# Autodesk Inventor assembly: COMPONENTS
(part 3 of 3)
701. RESC1005X35N_R198:1
702. RESC1005X35N_R199:1
703. RESC1005X35N_R200:1
704. RESC1005X35N_R155:1
705. RESC1005X35N_R156:1
706. RESC1005X35N_R225:1
707. RESC1005X35N_R228:1
708. RESC1005X35N_R229:1
709. RESC1005X35N_R230:1
710. RESC1005X35N_R231:1
711. RESC1005X35N_R232:1
712. RESC1005X35N_R233:1
713. RESC1005X35N_R234:1
714. RESC1005X35N_R168:1
715. RESC1005X35N_R181:1
716. RESC1005X35N_R17:1
717. RESC1005X35N_R18:1
718. RESC1005X35N_R37:1
719. RESC1005X35N_R38:1
720. RESC1005X35N_R57:1
721. RESC1005X35N_R58:1
722. RESC1005X35N_R19:1
723. RESC1005X35N_R39:1
724. RESC1005X35N_R59:1
725. RESC1005X35N_R20:1
726. RESC1005X35N_R40:1
727. RESC1005X35N_R60:1
728. RESC1005X35N_R209:1
729. RESC1005X35N_R220:1
730. RESC1005X35N_R61:1
731. RESC1005X35N_R65:1
732. RESC1005X35N_R67:1
733. RESC1005X35N_R62:1
734. RESC1005X35N_R64:1
735. RESC1005X35N_R63:1
736. RESC1005X35N_R66:1
737. RESC1005X35N_R70:1
738. RESC1005X35N_R71:1
739. RESC1005X35N_R72:1
740. RESC1005X35N_R73:1
741. RESC1005X35N_R75:1
742. RESC1005X35N_R76:1
743. RESC1005X35N_R77:1
744. RESC1005X35N_R91:1
745. RESC1005X35N_R92:1
746. RESC1005X35N_R94:1
747. RESC1005X35N_R95:1
748. RESC1005X35N_R80:1
749. RESC1005X35N_R81:1
750. RESC1005X35N_R82:1
751. RESC1005X35N_R83:1
752. RESC1005X35N_R84:1
753. RESC1005X35N_R86:1
754. RESC1005X35N_R90:1
755. RESC1005X35N_R93:1
756. RESC1005X35N_R99:1
757. RESC1005X35N_R85:1
758. RESC1005X35N_R87:1
759. RESC1005X35N_R407:1
760. RESC1005X35N_R408:1
761. RESC1608X50N_R441:1
762. RESC1608X50N_R440:1
763. RESC1608X50N_R439:1
764. RESC1608X50N_R435:1
765. RESC1608X50N_R101:1
766. RESC1608X50N_R107:1
767. RESC1608X50N_R108:1
768. RESC1608X50N_R78:1
769. RESC1608X50N_R79:1
770. RESC1608X50N_R88:1
771. RESC1608X50N_R89:1
772. RESC1608X50N_R98:1
773. RESC1608X50N_R192:1
774. RESC1608X50N_R193:1
775. RESC1608X50N_R149:1
776. RESC1608X50N_R153:1
777. RESC1608X50N_R68:1
778. RESC1608X50N_R69:1
779. RESC3216X70N_R460:1
780. RESC3216X70N_R165:1
781. RESC3216X70N_R74:1
782. RESC3216X70N_R474:1
783. TP107_GNDTP6:1
784. TP107_GNDTP5:1
785. TP107_GNDTP4:1
786. TP107_GNDTP3:1
787. TP107_GNDTP2:1
788. TP107_GNDTP1:1
789. TP107_TP1:1
790. TP107_TP4:1
791. TP107_TP5:1
792. TP107_TP10:1
793. TP107_TP6:1
794. TP107_TP8:1
795. TP107_TP11:1
796. TP107_TP7:1
797. TP107_TP9:1
798. DFN127P600X800X100-9T526X490N_U43:1
799. SOP65P640X120-24L25N_U71:1
800. TECONN_1734753-1_J10:1
